# Autodesk Inventor assembly: EX_ONE
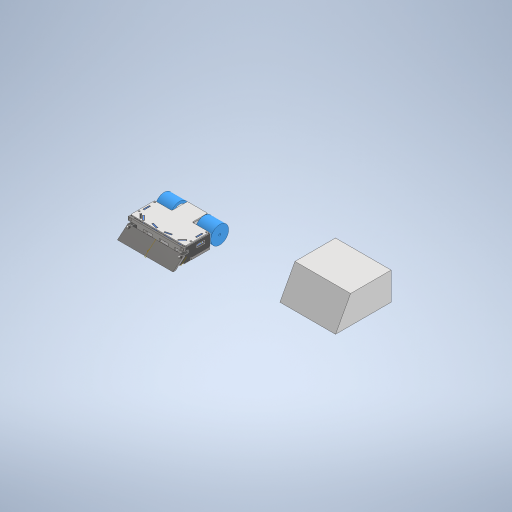
[picture p0: Inventor's stored thumbnail of the model, 512x512]
Saved by Autodesk Inventor 2023 (Build 270158000, 158)
## iProperties
Created: 2025-01-11
Part Number: EX_ONE
Document SubType Name: Assembly
Designer: kamil
Author: kamil
## Documents named in this file (18)
- C:\Users\kamil\Documents\PROJECTS - repos\EX_ONE_minisumo\mechanics\inventor_parts\EX_ONE.iam
- C:\Users\kamil\Documents\PROJECTS - repos\EX_ONE_minisumo\mechanics\inventor_parts\faulhaber_motor.ipt
- C:\Users\kamil\Documents\PROJECTS - repos\EX_ONE_minisumo\mechanics\inventor_parts\motors_mount.ipt
- C:\Users\kamil\Documents\PROJECTS - repos\EX_ONE_minisumo\mechanics\inventor_parts\kolo_tetsowe.ipt
- C:\Users\kamil\Documents\PROJECTS - repos\EX_ONE_minisumo\mechanics\inventor_parts\podstawa.ipt
- C:\Users\kamil\Documents\PROJECTS - repos\EX_ONE_minisumo\mechanics\inventor_parts\nóź.ipt
- C:\Users\kamil\Documents\PROJECTS - repos\EX_ONE_minisumo\mechanics\inventor_parts\TOF_VL53L0X (1).ipt
- C:\Users\kamil\Documents\PROJECTS - repos\EX_ONE_minisumo\mechanics\inventor_parts\pcb_pre.ipt
- C:\Users\kamil\Documents\PROJECTS - repos\EX_ONE_minisumo\mechanics\inventor_parts\minisunmo_testowe.ipt
- C:\Users\kamil\Documents\PROJECTS - repos\EX_ONE_minisumo\mechanics\inventor_parts\ściana.ipt
- C:\Users\kamil\Documents\PROJECTS - repos\EX_ONE_minisumo\mechanics\inventor_parts\ściana_MIR.ipt
- C:\Users\kamil\Documents\PROJECTS - repos\EX_ONE_minisumo\mechanics\inventor_parts\przod.ipt
- C:\Users\kamil\Documents\PROJECTS - repos\EX_ONE_minisumo\mechanics\inventor_parts\oslona.ipt
- C:\Users\kamil\Documents\PROJECTS - repos\EX_ONE_minisumo\mechanics\inventor_parts\pokrywa.ipt
- C:\Users\kamil\Documents\PROJECTS - repos\EX_ONE_minisumo\mechanics\inventor_parts\belka.ipt
- C:\Users\kamil\Documents\PROJECTS - repos\EX_ONE_minisumo\mechanics\inventor_parts\pcb_czujnik.ipt
- C:\Users\kamil\Documents\PROJECTS - repos\EX_ONE_minisumo\mechanics\inventor_parts\li_po_400mAh.ipt
- C:\Users\kamil\Documents\PROJECTS - repos\EX_ONE_minisumo\mechanics\inventor_parts\main_pcb.ipt
## Components (30 placed, 17 different names)
1. faulhaber_motor:1 — Równoległe:31, Zestawiające:31
2. faulhaber_motor:2 — Równoległe:32, Zestawiające:30
3. motors_mount:1 — Zestawiające:9, Zestawiające:29, Równoległe:31, Równoległe:32, Zestawiające:30, Zestawiające:31, Zestawiające:32, Zestawiające:33
4. kolo_tetsowe:1 — Zestawiające:33, Równoległe:33
5. nóź:1
6. kolo_tetsowe:2 — Zestawiające:9, Zestawiające:32, Równoległe:34
7. pcb_pre:1 — Zestawiające:11, Równoległe:18
8. TOF_VL53L0X (1):1 — Zestawiające:11, Równoległe:10, Równoległe:11, Równoległe:15, Równoległe:18, Równoległe:45, Równoległe:46
9. TOF_VL53L0X (1):2 — Równoległe:11, Równoległe:15, Równoległe:43, Równoległe:44
10. TOF_VL53L0X (1):3 — Równoległe:10, Równoległe:14, Kątowe:5, Równoległe:24, Zestawiające:21, Zestawiające:23, Równoległe:26, Kątowe:8, Kątowe:11, Równoległe:51
11. TOF_VL53L0X (1):5 — Równoległe:25, Zestawiające:24, Kątowe:7, Zestawiające:26, Kątowe:12, Równoległe:49
12. TOF_VL53L0X (1):6 — Równoległe:14, Kątowe:5, Równoległe:26, Zestawiające:25, Kątowe:8, Zestawiające:27, Kątowe:13, Równoległe:50
13. minisunmo_testowe:1
14. ściana:1 — Zestawiające:18, Równoległe:21, Zestawiające:19, Równoległe:22, Symetria:1, Zestawiające:28, Równoległe:27, Równoległe:28, Równoległe:29, Równoległe:30, Równoległe:33, Zestawiające:34, Kątowe:9, Równoległe:35, Zestawiające:35
15. ściana_MIR:1 — Symetria:1, Równoległe:34, Równoległe:36
16. przod:1 — Zestawiające:18, Równoległe:21, Zestawiające:19, Kątowe:6, Zestawiające:22, Zestawiające:23, Zestawiające:26, Zestawiające:27
17. oslona:1 — Równoległe:22, Zestawiające:41
18. pokrywa:1
19. TOF_VL53L0X (1):7 — Kątowe:6, Równoległe:24, Zestawiające:20, Zestawiające:22, Równoległe:25, Kątowe:7, Kątowe:10, Równoległe:47
20. belka:1 — Zestawiające:28, Równoległe:27, Równoległe:28
21. podstawa:1 — Zestawiające:29, Równoległe:29, Równoległe:30, Zestawiające:40
22. pcb_czujnik:1 — Zestawiające:34, Kątowe:9, Równoległe:35, Zestawiające:35
23. li_po_400mAh:1 — Zestawiające:40, Zestawiające:41
24. main_pcb:1 — Równoległe:36, Równoległe:37, 0, Równoległe:39, Równoległe:40, Równoległe:41, Równoległe:42, Zestawiające:36, Zestawiające:37, Zestawiające:38, Zestawiające:39
25. TOF_VL53L0X (1):8 — Równoległe:37, Równoległe:45, Równoległe:46
26. TOF_VL53L0X (1):9 — 0, Kątowe:12, Równoległe:49, Zestawiające:38
27. TOF_VL53L0X (1):10 — Równoległe:40, Kątowe:13, Zestawiające:39, Równoległe:50
28. TOF_VL53L0X (1):11 — Równoległe:39, Kątowe:10, Równoległe:47, Zestawiające:36
29. TOF_VL53L0X (1):12 — Równoległe:41, Kątowe:11, Zestawiające:37, Równoległe:51
30. TOF_VL53L0X (1):13 — Równoległe:42, Równoległe:43, Równoległe:44
## Relationships (70: Flush 34, Mate 26, Angle 9, Symmetry 1)
- Zestawiające:9 [Mate]: motors_mount:1 ↔ kolo_tetsowe:2
- Zestawiające:11 [Mate]: pcb_pre:1 ↔ TOF_VL53L0X (1):1
- Równoległe:10 [Flush]: TOF_VL53L0X (1):1 ↔ TOF_VL53L0X (1):3
- Równoległe:11 [Flush]: TOF_VL53L0X (1):1 ↔ TOF_VL53L0X (1):2
- Równoległe:14 [Flush]: TOF_VL53L0X (1):3 ↔ TOF_VL53L0X (1):6
- Równoległe:15 [Flush]: TOF_VL53L0X (1):1 ↔ TOF_VL53L0X (1):2
- Kątowe:5 [Angle] (30 deg): TOF_VL53L0X (1):3 ↔ TOF_VL53L0X (1):6
- Równoległe:18 [Flush] (2 mm): pcb_pre:1 ↔ TOF_VL53L0X (1):1
- Zestawiające:18 [Mate]: ściana:1 ↔ przod:1
- Równoległe:21 [Flush]: ściana:1 ↔ przod:1
- Zestawiające:19 [Mate]: ściana:1 ↔ przod:1
- Równoległe:22 [Flush]: ściana:1 ↔ oslona:1
- Kątowe:6 [Angle] (-195 deg): przod:1 ↔ TOF_VL53L0X (1):7
- Równoległe:24 [Flush]: TOF_VL53L0X (1):3 ↔ TOF_VL53L0X (1):7
- Symetria:1 [Symmetry]: ściana:1 ↔ ściana_MIR:1
- Zestawiające:20 [Mate] (10 mm): TOF_VL53L0X (1):7
- Zestawiające:21 [Mate] (-10 mm): TOF_VL53L0X (1):3
- Zestawiające:22 [Mate] (2 mm): przod:1 ↔ TOF_VL53L0X (1):7
- Zestawiające:23 [Mate] (2 mm): TOF_VL53L0X (1):3 ↔ przod:1
- Równoległe:25 [Flush]: TOF_VL53L0X (1):5 ↔ TOF_VL53L0X (1):7
- Równoległe:26 [Flush]: TOF_VL53L0X (1):3 ↔ TOF_VL53L0X (1):6
- Zestawiające:24 [Mate] (34 mm): TOF_VL53L0X (1):5
- Zestawiające:25 [Mate] (-34 mm): TOF_VL53L0X (1):6
- Kątowe:7 [Angle] (30 deg): TOF_VL53L0X (1):5 ↔ TOF_VL53L0X (1):7
- Kątowe:8 [Angle] (30 deg): TOF_VL53L0X (1):3 ↔ TOF_VL53L0X (1):6
- Zestawiające:26 [Mate] (5 mm): TOF_VL53L0X (1):5 ↔ przod:1
- Zestawiające:27 [Mate] (5 mm): TOF_VL53L0X (1):6 ↔ przod:1
- Zestawiające:28 [Mate]: ściana:1 ↔ belka:1
- Równoległe:27 [Flush]: ściana:1 ↔ belka:1
- Równoległe:28 [Flush]: ściana:1 ↔ belka:1
- Zestawiające:29 [Mate]: motors_mount:1 ↔ podstawa:1
- Równoległe:29 [Flush]: ściana:1 ↔ podstawa:1
- Równoległe:30 [Flush]: ściana:1 ↔ podstawa:1
- Równoległe:31 [Flush]: faulhaber_motor:1 ↔ motors_mount:1
- Równoległe:32 [Flush]: faulhaber_motor:2 ↔ motors_mount:1
- Zestawiające:30 [Mate]: faulhaber_motor:2 ↔ motors_mount:1
- Zestawiające:31 [Mate]: faulhaber_motor:1 ↔ motors_mount:1
- Zestawiające:32 [Mate]: motors_mount:1 ↔ kolo_tetsowe:2
- Zestawiające:33 [Mate]: motors_mount:1 ↔ kolo_tetsowe:1
- Równoległe:33 [Flush]: kolo_tetsowe:1 ↔ ściana:1
- Równoległe:34 [Flush]: kolo_tetsowe:2 ↔ ściana_MIR:1
- Zestawiające:34 [Mate]: ściana:1 ↔ pcb_czujnik:1
- Kątowe:9 [Angle] (0 deg): ściana:1 ↔ pcb_czujnik:1
- Równoległe:35 [Flush]: ściana:1 ↔ pcb_czujnik:1
- Zestawiające:35 [Mate] (0.5 mm): ściana:1 ↔ pcb_czujnik:1
- Równoległe:36 [Flush]: ściana_MIR:1 ↔ main_pcb:1
- Równoległe:37 [Flush]: main_pcb:1 ↔ TOF_VL53L0X (1):8
- 0 [Flush]: main_pcb:1 ↔ TOF_VL53L0X (1):9
- Równoległe:39 [Flush]: main_pcb:1 ↔ TOF_VL53L0X (1):11
- Równoległe:40 [Flush]: main_pcb:1 ↔ TOF_VL53L0X (1):10
- Równoległe:41 [Flush]: main_pcb:1 ↔ TOF_VL53L0X (1):12
- Równoległe:42 [Flush]: main_pcb:1 ↔ TOF_VL53L0X (1):13
- Równoległe:43 [Flush]: TOF_VL53L0X (1):2 ↔ TOF_VL53L0X (1):13
- Równoległe:44 [Flush]: TOF_VL53L0X (1):2 ↔ TOF_VL53L0X (1):13
- Równoległe:45 [Flush]: TOF_VL53L0X (1):1 ↔ TOF_VL53L0X (1):8
- Równoległe:46 [Flush]: TOF_VL53L0X (1):1 ↔ TOF_VL53L0X (1):8
- Kątowe:10 [Angle] (0 deg): TOF_VL53L0X (1):7 ↔ TOF_VL53L0X (1):11
- Równoległe:47 [Flush]: TOF_VL53L0X (1):7 ↔ TOF_VL53L0X (1):11
- Kątowe:11 [Angle] (0 deg): TOF_VL53L0X (1):3 ↔ TOF_VL53L0X (1):12
- Zestawiające:36 [Mate] (-2 mm): main_pcb:1 ↔ TOF_VL53L0X (1):11
- Zestawiające:37 [Mate] (-2 mm): main_pcb:1 ↔ TOF_VL53L0X (1):12
- Kątowe:12 [Angle] (0 deg): TOF_VL53L0X (1):5 ↔ TOF_VL53L0X (1):9
- Równoległe:49 [Flush]: TOF_VL53L0X (1):5 ↔ TOF_VL53L0X (1):9
- Zestawiające:38 [Mate] (-2 mm): main_pcb:1 ↔ TOF_VL53L0X (1):9
- Kątowe:13 [Angle] (0 deg): TOF_VL53L0X (1):6 ↔ TOF_VL53L0X (1):10
- Zestawiające:39 [Mate] (-2 mm): main_pcb:1 ↔ TOF_VL53L0X (1):10
- Równoległe:50 [Flush]: TOF_VL53L0X (1):6 ↔ TOF_VL53L0X (1):10
- Równoległe:51 [Flush]: TOF_VL53L0X (1):3 ↔ TOF_VL53L0X (1):12
- Zestawiające:40 [Mate]: podstawa:1 ↔ li_po_400mAh:1
- Zestawiające:41 [Mate]: oslona:1 ↔ li_po_400mAh:1
